# Autodesk Inventor assembly: Track Design 9-24-19
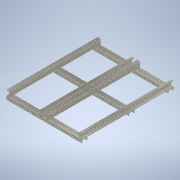
[picture p0: Inventor's stored thumbnail of the model, 180x180]
Saved by Autodesk Inventor 2020 (Build 240168000, 168)
## iProperties
Created: 2019-07-25
Part Number: Track Design 9-24-19
Document SubType Name: Assembly
Designer: Corey
Author: Corey
## Documents named in this file (3)
- C:\Users\spenc\OneDrive\Desktop\Vex Robotics\Tower-Takeover-CAD\Track Design 9-24-19.iam
- C:\Users\spenc\OneDrive\Desktop\Vex Robotics\Tower-Takeover-CAD\Parts\Structure\C-Channels\Aluminum\2-Wide\Aluminum C-Channel 1x2x1x35.ipt
- C:\Users\spenc\OneDrive\Desktop\Vex Robotics\Tower-Takeover-CAD\Parts\Structure\C-Channels\Aluminum\2-Wide\Aluminum C-Channel 1x2x1x29.ipt
## Components (7 placed, 2 different names)
1. Aluminum C-Channel 1x2x1x35:2 — Flush:24
2. Aluminum C-Channel 1x2x1x35:3
3. Aluminum C-Channel 1x2x1x35:4 — Mate:9
4. Aluminum C-Channel 1x2x1x35:5 — Mate:7, Flush:20, Flush:21, Mate:8, Flush:22, Flush:23
5. Aluminum C-Channel 1x2x1x29:1 — Mate:8, Flush:22, Flush:23
6. Aluminum C-Channel 1x2x1x29:2 — Mate:7, Flush:20, Flush:21
7. Aluminum C-Channel 1x2x1x29:3 — Mate:9, Flush:24
## Relationships (8: Flush 5, Mate 3)
- Mate:7: Aluminum C-Channel 1x2x1x35:5 ↔ Aluminum C-Channel 1x2x1x29:2
- Flush:20: Aluminum C-Channel 1x2x1x35:5 ↔ Aluminum C-Channel 1x2x1x29:2
- Flush:21: Aluminum C-Channel 1x2x1x35:5 ↔ Aluminum C-Channel 1x2x1x29:2
- Mate:8: Aluminum C-Channel 1x2x1x35:5 ↔ Aluminum C-Channel 1x2x1x29:1
- Flush:22: Aluminum C-Channel 1x2x1x35:5 ↔ Aluminum C-Channel 1x2x1x29:1
- Flush:23: Aluminum C-Channel 1x2x1x35:5 ↔ Aluminum C-Channel 1x2x1x29:1
- Mate:9: Aluminum C-Channel 1x2x1x35:4 ↔ Aluminum C-Channel 1x2x1x29:3
- Flush:24: Aluminum C-Channel 1x2x1x35:2 ↔ Aluminum C-Channel 1x2x1x29:3
